# Autodesk Inventor assembly: Right Structure
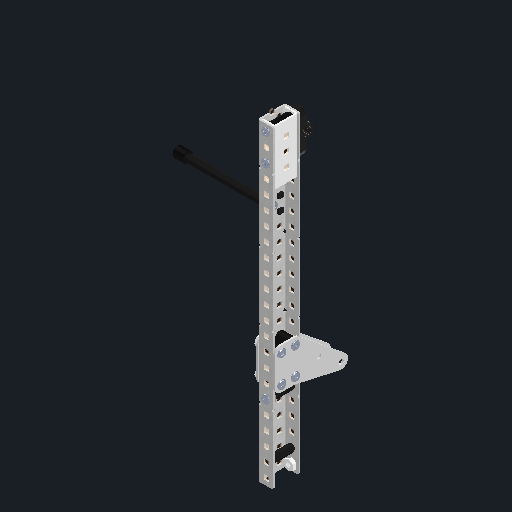
[picture p0: Inventor's stored thumbnail of the model, 512x512]
Saved by Autodesk Inventor 2025 (Build 290162000, 162)
## iProperties
Created: 2024-10-20
Part Number: Right Structure
Document SubType Name: Assembly
Designer: Averey Ku
Author: Averey Ku
## Documents named in this file (27)
- D:\VEX\High Stakes\CAD\V2\Tower\Right Structure\Right Structure.iam
- D:\VEX\High Stakes\CAD\V2\Tower\Right Structure\Right Alu C 1x2x1x23.ipt
- D:\VEX\High Stakes\CAD\ROBOPROS-CAD-Inventor\Structure\Standoff\Standoff .75.ipt
- D:\VEX\High Stakes\CAD\ROBOPROS-CAD-Inventor\Motion\Spacers\Washer Steel\SWasher .375 OD x .062500.ipt
- D:\VEX\High Stakes\CAD\ROBOPROS-CAD-Inventor\Structure\Hardware\Screw Steel - Star\SScrew Star Smooth .290.ipt
- D:\VEX\High Stakes\CAD\ROBOPROS-CAD-Inventor\Structure\Standoff\Standoff .875.ipt
- D:\VEX\High Stakes\CAD\ROBOPROS-CAD-Inventor\Structure\Hardware\Nut Nylon\Nut Nylon - White.ipt
- D:\VEX\High Stakes\CAD\V2\Tower\Right Structure\Right HS Pillow Bearing Block.ipt
- D:\VEX\High Stakes\CAD\V2\Tower\Right Structure\Right C Channel Coupler.ipt
- D:\VEX\High Stakes\CAD\ROBOPROS-CAD-Inventor\Structure\Hardware\Screw Shoulder Robosource\SScrew Shoulder Smooth .375 x .12.ipt
- D:\VEX\High Stakes\CAD\ROBOPROS-CAD-Inventor\Structure\Hardware\Screw Steel - Star\SScrew Star Smooth 1.250.ipt
- D:\VEX\High Stakes\CAD\ROBOPROS-CAD-Inventor\Motion\Spacers\Spacer Nylon .375 OD\NSpacer .375 OD x .250.ipt
- D:\VEX\High Stakes\CAD\ROBOPROS-CAD-Inventor\Motion\Spacers\Spacer Nylon .375 OD\NSpacer .375 OD x .500.ipt
- D:\VEX\High Stakes\CAD\V2\Tower\Right Structure\Right Angle Brace Gusset.ipt
- D:\VEX\High Stakes\CAD\ROBOPROS-CAD-Inventor\Structure\Standoff\Standoff .50.ipt
- D:\VEX\High Stakes\CAD\ROBOPROS-CAD-Inventor\Structure\Hardware\Screw Shoulder Robosource\SScrew Shoulder Smooth .290 x .09.ipt
- D:\VEX\High Stakes\CAD\ROBOPROS-CAD-Inventor\Structure\Hardware\Screw Shoulder Robosource\SScrew Shoulder Smooth .500 x .04.ipt
- D:\VEX\High Stakes\CAD\ROBOPROS-CAD-Inventor\Structure\Standoff\Standoff 3.00.ipt
- D:\VEX\High Stakes\CAD\V2\Tower\Right Structure\Right 4-Post Standoff Retainer.ipt
- D:\VEX\High Stakes\CAD\ROBOPROS-CAD-Inventor\Structure\Hardware\Screw Steel - Star\SScrew Star Smooth .875.ipt
- D:\VEX\High Stakes\CAD\ROBOPROS-CAD-Inventor\Motion\Spacers\Spacer Nylon .375 OD\NSpacer .375 OD x .375.ipt
- C:\Users\avere\VEX\High Stakes\CAD\ROBOPROS-CAD-Inventor\Structure\Standoff.ipt
- C:\Users\avere\VEX\High Stakes\CAD\ROBOPROS-CAD-Inventor\Motion\Spacers\Washer Steel.ipt
- C:\Users\avere\VEX\High Stakes\CAD\ROBOPROS-CAD-Inventor\Structure\Hardware\Screw Steel - Star.ipt
- C:\Users\avere\VEX\High Stakes\CAD\ROBOPROS-CAD-Inventor\Structure\Hardware\Nut Nylon.ipt
- C:\Users\avere\VEX\High Stakes\CAD\ROBOPROS-CAD-Inventor\Structure\Hardware\Screw Shoulder Robosource.ipt
- C:\Users\avere\VEX\High Stakes\CAD\ROBOPROS-CAD-Inventor\Motion\Spacers\Spacer Nylon .375 OD.ipt
## Components (37 placed, 20 different names)
1. Right Alu C 1x2x1x23:1 — Mate:6, Insert:1, Insert:3, Insert:4, Insert:5, Mate:1, Insert:6, Insert:7, Insert:8, Mate:2, Insert:16, Insert:15, Insert:17, Mate:3, Insert:18, Mate:4, Insert:25, Insert:26, Mate:5
2. Standoff .75:1 — Insert:1, Insert:2
3. SWasher .375 OD x .062500:1 — Insert:2
4. SScrew Star Smooth .290:1 — Insert:6
5. Standoff .875:2 — Insert:3
6. Nut Nylon - White:1 — Insert:4
7. Right HS Pillow Bearing Block:1 — Insert:5, Mate:1, Insert:10, Insert:9
8. Right C Channel Coupler:1 — Insert:8, Mate:2, Insert:12, Insert:14
9. SScrew Shoulder Smooth .375 x .12:1 — Insert:7
10. SScrew Star Smooth 1.250:2 — Insert:15
11. Nut Nylon - White:2 — Insert:10
12. Nut Nylon - White:3 — Insert:9
13. NSpacer .375 OD x .250:1 — Insert:12, Insert:11
14. NSpacer .375 OD x .500:2 — Insert:11
15. NSpacer .375 OD x .250:3 — Insert:13
16. NSpacer .375 OD x .500:4 — Insert:14, Insert:13
17. SScrew Star Smooth 1.250:3 — Insert:16
18. Right Angle Brace Gusset:1 — Insert:17, Mate:3, Insert:19, Insert:20, Insert:22, Insert:21, Insert:24, Insert:30
19. Right Angle Brace Gusset:2 — Insert:18, Mate:4, Insert:23, Insert:31
20. NSpacer .375 OD x .500:5 — Insert:19
21. NSpacer .375 OD x .500:6 — Insert:20
22. Standoff .50:3 — Insert:22
23. NSpacer .375 OD x .500:7 — Insert:21
24. SScrew Shoulder Smooth .375 x .12:2 — Insert:23
25. SScrew Shoulder Smooth .290 x .09:3 — Insert:24
26. SScrew Shoulder Smooth .500 x .04:4 — Insert:25
27. Standoff 3.00:4 — Insert:29, Insert:32
28. Right 4-Post Standoff Retainer:1 — Insert:29, Insert:26, Mate:5
29. NSpacer .375 OD x .375:8 — Insert:32
30. Nut Nylon - White:4 — Insert:31
31. SScrew Star Smooth .875:4 — Insert:30
32. Nut Nylon - White:5
33. SScrew Star Smooth .875:5
34. Nut Nylon - White:6
35. SScrew Star Smooth .875:6
36. Nut Nylon - White:7
37. SScrew Star Smooth .875:7
## Component patterns: (4 elements, first: Nut Nylon - White:4 + SScrew Star Smooth .875:4)
## Relationships (36: Insert 30, Mate 6)
- Mate:6: Right Alu C 1x2x1x23:1
- Insert:1: Right Alu C 1x2x1x23:1 ↔ Standoff .75:1
- Insert:2: Standoff .75:1 ↔ SWasher .375 OD x .062500:1
- Insert:3: Right Alu C 1x2x1x23:1 ↔ Standoff .875:2
- Insert:4: Right Alu C 1x2x1x23:1 ↔ Nut Nylon - White:1
- Insert:5: Right Alu C 1x2x1x23:1 ↔ Right HS Pillow Bearing Block:1
- Mate:1: Right Alu C 1x2x1x23:1 ↔ Right HS Pillow Bearing Block:1
- Insert:6: Right Alu C 1x2x1x23:1 ↔ SScrew Star Smooth .290:1
- Insert:7: Right Alu C 1x2x1x23:1 ↔ SScrew Shoulder Smooth .375 x .12:1
- Insert:8: Right Alu C 1x2x1x23:1 ↔ Right C Channel Coupler:1
- Mate:2: Right Alu C 1x2x1x23:1 ↔ Right C Channel Coupler:1
- Insert:10: Right HS Pillow Bearing Block:1 ↔ Nut Nylon - White:2
- Insert:9: Right HS Pillow Bearing Block:1 ↔ Nut Nylon - White:3
- Insert:12: Right C Channel Coupler:1 ↔ NSpacer .375 OD x .250:1
- Insert:11: NSpacer .375 OD x .250:1 ↔ NSpacer .375 OD x .500:2
- Insert:14: Right C Channel Coupler:1 ↔ NSpacer .375 OD x .500:4
- Insert:13: NSpacer .375 OD x .250:3 ↔ NSpacer .375 OD x .500:4
- Insert:16: Right Alu C 1x2x1x23:1 ↔ SScrew Star Smooth 1.250:3
- Insert:15: Right Alu C 1x2x1x23:1 ↔ SScrew Star Smooth 1.250:2
- Insert:17 (12.7 mm): Right Alu C 1x2x1x23:1 ↔ Right Angle Brace Gusset:1
- Mate:3: Right Alu C 1x2x1x23:1 ↔ Right Angle Brace Gusset:1
- Insert:18: Right Alu C 1x2x1x23:1 ↔ Right Angle Brace Gusset:2
- Mate:4: Right Alu C 1x2x1x23:1 ↔ Right Angle Brace Gusset:2
- Insert:19: Right Angle Brace Gusset:1 ↔ NSpacer .375 OD x .500:5
- Insert:20: Right Angle Brace Gusset:1 ↔ NSpacer .375 OD x .500:6
- Insert:22: Right Angle Brace Gusset:1 ↔ Standoff .50:3
- Insert:21: Right Angle Brace Gusset:1 ↔ NSpacer .375 OD x .500:7
- Insert:23: Right Angle Brace Gusset:2 ↔ SScrew Shoulder Smooth .375 x .12:2
- Insert:24: Right Angle Brace Gusset:1 ↔ SScrew Shoulder Smooth .290 x .09:3
- Insert:25: Right Alu C 1x2x1x23:1 ↔ SScrew Shoulder Smooth .500 x .04:4
- Insert:29: Standoff 3.00:4 ↔ Right 4-Post Standoff Retainer:1
- Insert:26: Right Alu C 1x2x1x23:1 ↔ Right 4-Post Standoff Retainer:1
- Mate:5: Right Alu C 1x2x1x23:1 ↔ Right 4-Post Standoff Retainer:1
- Insert:31: Right Angle Brace Gusset:2 ↔ Nut Nylon - White:4
- Insert:30: Right Angle Brace Gusset:1 ↔ SScrew Star Smooth .875:4
- Insert:32: Standoff 3.00:4 ↔ NSpacer .375 OD x .375:8
